# Autodesk Inventor assembly: robot-podvozek
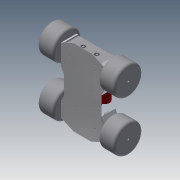
[picture p0: Inventor's stored thumbnail of the model, 180x180]
Saved by Autodesk Inventor 2013 (Build 170138000, 138)
## iProperties
Created: 2012-08-13
Part Number: robot-podvozek
Document SubType Name: Assembly
Designer: Petr
Author: Petr
## Documents named in this file (18)
- C:\Users\Petr\Documents\Inventor\robot-podvozek\robot-podvozek.iam
- C:\Users\Petr\Documents\Inventor\robot-podvozek\hridel.ipt
- C:\Users\Petr\Documents\Inventor\robot-podvozek\hridel kuzelova kolecka.ipt
- C:\Users\Petr\Documents\Inventor\robot-podvozek\drzak_motory.ipt
- C:\Users\Petr\Documents\Inventor\robot-podvozek\gear motor.ipt
- C:\Users\Petr\Documents\Inventor\robot-podvozek\gear hridel.ipt
- C:\Users\Petr\Documents\Inventor\robot-podvozek\robot-podvozek\Design Accelerator\Spur Gears3.iam
- C:\Users\Petr\Documents\Inventor\robot-podvozek\robot-podvozek\Design Accelerator\Spur Gears4.iam
- C:\Users\Petr\Documents\Inventor\robot-podvozek\prepazka.ipt
- C:\Users\Petr\Documents\Inventor\robot-podvozek\prepazka_kola.ipt
- C:\Users\Petr\Documents\Inventor\robot-podvozek\podvozek.ipt
- C:\Users\Petr\Documents\Inventor\robot-podvozek\zadni_strana.ipt
- C:\Users\Petr\Documents\Inventor\robot-podvozek\predni strana.ipt
- C:\Users\Petr\Documents\Inventor\robotic arm\rameno\robotic_arm.iam
- C:\Users\Petr\Documents\Inventor\robot-podvozek\kolo.ipt
- C:\Users\Petr\Documents\Inventor\robot-podvozek\podvozek_dibond.ipt
- C:\Users\Petr\Documents\Inventor\robot-podvozek\podvozek_priklopny_kryt.ipt
- C:\Users\Petr\Documents\Inventor\robot-podvozek\DC_motor_with_encoder.ipt
## Components (37 placed, 16 different names)
1. hridel:1 — Mate:1, Flush:1, Mate:3, Flush:2, Mate:4, Mate:5, Flush:3, Mate:6, Mate:16, Mate:21, Flush:23, Mate:82
2. hridel:2 — Mate:1, Flush:1, Flush:4, Mate:7, Mate:8, Flush:5, Mate:9, Mate:10, Mate:16, Flush:24, Mate:22, Mate:29, Mate:30, Mate:31, Mate:32, Mate:33, Mate:34, Mate:35, Mate:36
3. hridel kuzelova kolecka:1 — Mate:3, Flush:2, Mate:4, Mate:12, Flush:8, Flush:9
4. hridel kuzelova kolecka:2 — Flush:4, Mate:7, Mate:8, Flush:12, Flush:13, Mate:14, Mate:37
5. hridel kuzelova kolecka:3 — Flush:5, Mate:9, Mate:10, Flush:10, Flush:11, Mate:13
6. hridel kuzelova kolecka:4 — Mate:5, Flush:3, Mate:6, Mate:11, Flush:6, Flush:7, Mate:38
7. hridel kuzelova kolecka:5 — Mate:11, Flush:6, Flush:7, Mate:45, Mate:46, Mate:47
8. hridel kuzelova kolecka:6 — Flush:10, Flush:11, Mate:13, Mate:48, Mate:49, Mate:50
9. hridel kuzelova kolecka:7 — Flush:12, Flush:13, Mate:14, Mate:39, Mate:40, Mate:41
10. hridel kuzelova kolecka:8 — Mate:12, Flush:8, Flush:9, Mate:42, Mate:43, Mate:44
11. drzak_motory:1 — Mate:15, Flush:14, Mate:85, Mate:86, Mate:88, Mate:89, Mate:90
12. gear motor:1 — Mate:23, Mate:24, Mate:82, Mate:83
13. gear motor:2 — Mate:26, Mate:27
14. gear hridel:1 — Mate:21, Flush:23, Mate:25, Mate:52, Mate:84
15. gear hridel:2 — Flush:24, Mate:22, Mate:28, Mate:91
16. Spur Gears:1 [sub-assembly] — Mate:23, Mate:24, Mate:25, Mate:84
17. Spur Gears:2 [sub-assembly] — Mate:26, Mate:27, Mate:28, Mate:91
18. prepazka:1 — Mate:29, Mate:30, Mate:37
19. prepazka:2 — Mate:31, Mate:32, Flush:28, Mate:52, Flush:30, Flush:31, Flush:32, Mate:74
20. prepazka:3 — Mate:33, Mate:34, Mate:38
21. prepazka:4 — Mate:35, Mate:36, Flush:27, Mate:51, Mate:71
22. prepazka_kola:1 — Mate:39, Mate:40, Mate:41
23. prepazka_kola:2 — Mate:48, Mate:49, Mate:50
24. prepazka_kola:3 — Mate:45, Mate:46, Mate:47, Flush:27, Mate:51
25. prepazka_kola:4 — Mate:42, Mate:43, Mate:44, Flush:28
26. podvozek:1 — Flush:30, Flush:31, Flush:32, Flush:33, Flush:34, Mate:55, Flush:35, Flush:36, Mate:56, Mate:57, Mate:78, Mate:79
27. zadni_strana:1 — Flush:33, Flush:34, Flush:36, Mate:63, Mate:65, Mate:67, Mate:68, Mate:72
28. predni strana:1 — Mate:55, Flush:35, Mate:56, Mate:57, Mate:64, Mate:66, Mate:69, Mate:70, Mate:73
29. robotic_arm:1 [sub-assembly] — Mate:77, Mate:78, Mate:79
30. kolo:1 — Mate:63, Mate:68
31. kolo:2 — Mate:64, Mate:70
32. kolo:3 — Mate:65, Mate:67
33. kolo:4 — Mate:66, Mate:69
34. podvozek_dibond:1 — Mate:71, Mate:72, Mate:73, Mate:75, Mate:76, Mate:77
35. podvozek_priklopny_kryt:1 — Mate:74, Mate:75, Mate:76
36. DC_motor_with_encoder:1 — Mate:83, Mate:85, Mate:86
37. DC_motor_with_encoder:2 — Mate:88, Mate:89, Mate:90
## Relationships (101: Mate 76, Flush 25)
- Mate:1: hridel:1 ↔ hridel:2
- Flush:1: hridel:1 ↔ hridel:2
- Mate:3: hridel:1 ↔ hridel kuzelova kolecka:1
- Flush:2: hridel:1 ↔ hridel kuzelova kolecka:1
- Mate:4 (189.5 mm): hridel:1 ↔ hridel kuzelova kolecka:1
- Mate:5: hridel:1 ↔ hridel kuzelova kolecka:4
- Flush:3: hridel:1 ↔ hridel kuzelova kolecka:4
- Mate:6 (11.2 mm): hridel:1 ↔ hridel kuzelova kolecka:4
- Flush:4: hridel:2 ↔ hridel kuzelova kolecka:2
- Mate:7: hridel:2 ↔ hridel kuzelova kolecka:2
- Mate:8 (189.5 mm): hridel:2 ↔ hridel kuzelova kolecka:2
- Flush:5: hridel:2 ↔ hridel kuzelova kolecka:3
- Mate:9: hridel:2 ↔ hridel kuzelova kolecka:3
- Mate:10 (11.2 mm): hridel:2 ↔ hridel kuzelova kolecka:3
- Mate:11 (16 mm): hridel kuzelova kolecka:4 ↔ hridel kuzelova kolecka:5
- Flush:6: hridel kuzelova kolecka:4 ↔ hridel kuzelova kolecka:5
- Flush:7 (-16 mm): hridel kuzelova kolecka:4 ↔ hridel kuzelova kolecka:5
- Mate:12 (16 mm): hridel kuzelova kolecka:1 ↔ hridel kuzelova kolecka:8
- Flush:8: hridel kuzelova kolecka:1 ↔ hridel kuzelova kolecka:8
- Flush:9 (16 mm): hridel kuzelova kolecka:1 ↔ hridel kuzelova kolecka:8
- Flush:10 (-16 mm): hridel kuzelova kolecka:3 ↔ hridel kuzelova kolecka:6
- Flush:11: hridel kuzelova kolecka:3 ↔ hridel kuzelova kolecka:6
- Mate:13 (16 mm): hridel kuzelova kolecka:3 ↔ hridel kuzelova kolecka:6
- Flush:12 (-16 mm): hridel kuzelova kolecka:2 ↔ hridel kuzelova kolecka:7
- Flush:13: hridel kuzelova kolecka:2 ↔ hridel kuzelova kolecka:7
- Mate:14 (16 mm): hridel kuzelova kolecka:2 ↔ hridel kuzelova kolecka:7
- Mate:15 (24.1 mm): drzak_motory:1
- Flush:14: drzak_motory:1
- Mate:16 (48.2 mm): hridel:1 ↔ hridel:2
- Mate:21: hridel:1 ↔ gear hridel:1
- Flush:23: hridel:1 ↔ gear hridel:1
- Flush:24: hridel:2 ↔ gear hridel:2
- Mate:22: hridel:2 ↔ gear hridel:2
- Mate:23: gear motor:1 ↔ Spur Gears:1
- Mate:24: gear motor:1 ↔ Spur Gears:1
- Mate:25: gear hridel:1 ↔ Spur Gears:1
- Mate:26: gear motor:2 ↔ Spur Gears:2
- Mate:27: gear motor:2 ↔ Spur Gears:2
- Mate:28: gear hridel:2 ↔ Spur Gears:2
- Mate:29 (24.1 mm): hridel:2 ↔ prepazka:1
- Mate:30: hridel:2 ↔ prepazka:1
- Mate:31 (24.1 mm): hridel:2 ↔ prepazka:2
- Mate:32: hridel:2 ↔ prepazka:2
- Mate:33 (24.1 mm): hridel:2 ↔ prepazka:3
- Mate:34: hridel:2 ↔ prepazka:3
- Mate:35 (24.1 mm): hridel:2 ↔ prepazka:4
- Mate:36: hridel:2 ↔ prepazka:4
- Mate:37 (-0.5 mm): hridel kuzelova kolecka:2 ↔ prepazka:1
- Mate:38 (-0.5 mm): hridel kuzelova kolecka:4 ↔ prepazka:3
- Mate:39: hridel kuzelova kolecka:7 ↔ prepazka_kola:1
- Mate:40: hridel kuzelova kolecka:7 ↔ prepazka_kola:1
- Mate:41 (-0.5 mm): hridel kuzelova kolecka:7 ↔ prepazka_kola:1
- Mate:42: hridel kuzelova kolecka:8 ↔ prepazka_kola:4
- Mate:43: hridel kuzelova kolecka:8 ↔ prepazka_kola:4
- Mate:44 (-0.5 mm): hridel kuzelova kolecka:8 ↔ prepazka_kola:4
- Mate:45: hridel kuzelova kolecka:5 ↔ prepazka_kola:3
- Mate:46: hridel kuzelova kolecka:5 ↔ prepazka_kola:3
- Mate:47 (-0.5 mm): hridel kuzelova kolecka:5 ↔ prepazka_kola:3
- Mate:48: hridel kuzelova kolecka:6 ↔ prepazka_kola:2
- Mate:49: hridel kuzelova kolecka:6 ↔ prepazka_kola:2
- Mate:50 (-0.5 mm): hridel kuzelova kolecka:6 ↔ prepazka_kola:2
- Flush:27 (-26.5 mm): prepazka:4 ↔ prepazka_kola:3
- Mate:51: prepazka:4 ↔ prepazka_kola:3
- Flush:28 (-26.5 mm): prepazka:2 ↔ prepazka_kola:4
- Mate:52 (-11 mm): gear hridel:1 ↔ prepazka:2
- Flush:30: prepazka:2 ↔ podvozek:1
- Flush:31 (-27 mm): prepazka:2 ↔ podvozek:1
- Flush:32 (-62.65 mm): prepazka:2 ↔ podvozek:1
- Flush:33 (2 mm): podvozek:1 ↔ zadni_strana:1
- Flush:34: podvozek:1 ↔ zadni_strana:1
- Mate:55: podvozek:1 ↔ predni strana:1
- Flush:35 (2 mm): podvozek:1 ↔ predni strana:1
- Flush:36 (-78.9 mm): podvozek:1 ↔ zadni_strana:1
- Mate:56: podvozek:1 ↔ predni strana:1
- Mate:57 (-89.15 mm): podvozek:1 ↔ predni strana:1
- Mate:63: zadni_strana:1 ↔ kolo:1
- Mate:64: predni strana:1 ↔ kolo:2
- Mate:65: zadni_strana:1 ↔ kolo:3
- Mate:66: predni strana:1 ↔ kolo:4
- Mate:67 (4 mm): zadni_strana:1 ↔ kolo:3
- Mate:68 (4 mm): zadni_strana:1 ↔ kolo:1
- Mate:69 (4 mm): predni strana:1 ↔ kolo:4
- Mate:70 (4 mm): predni strana:1 ↔ kolo:2
- Mate:71: prepazka:4 ↔ podvozek_dibond:1
- Mate:72: zadni_strana:1 ↔ podvozek_dibond:1
- Mate:73: predni strana:1 ↔ podvozek_dibond:1
- Mate:74: prepazka:2 ↔ podvozek_priklopny_kryt:1
- Mate:75: podvozek_dibond:1 ↔ podvozek_priklopny_kryt:1
- Mate:76: podvozek_dibond:1 ↔ podvozek_priklopny_kryt:1
- Mate:77 (30 mm): robotic_arm:1 ↔ podvozek_dibond:1
- Mate:78: podvozek:1 ↔ robotic_arm:1
- Mate:79: podvozek:1 ↔ robotic_arm:1
- Mate:82 (27.2 mm): hridel:1 ↔ gear motor:1
- Mate:83: gear motor:1 ↔ DC_motor_with_encoder:1
- Mate:84: gear hridel:1 ↔ Spur Gears:1
- Mate:85 (1.2 mm): drzak_motory:1 ↔ DC_motor_with_encoder:1
- Mate:86: drzak_motory:1 ↔ DC_motor_with_encoder:1
- Mate:88: drzak_motory:1 ↔ DC_motor_with_encoder:2
- Mate:89: drzak_motory:1 ↔ DC_motor_with_encoder:2
- Mate:90 (1.2 mm): drzak_motory:1 ↔ DC_motor_with_encoder:2
- Mate:91: gear hridel:2 ↔ Spur Gears:2
